# Autodesk Inventor assembly: Ensamblaje1
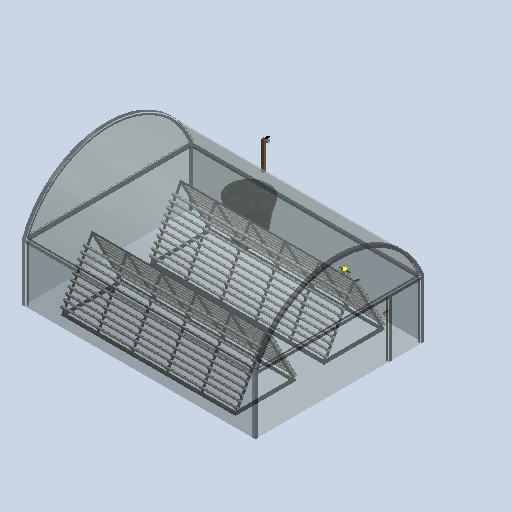
[picture p0: Inventor's stored thumbnail of the model, 512x512]
Saved by Autodesk Inventor 2026.1 (Build 301233020, 233B)
## iProperties
Created: 2025-11-02
Part Number: Ensamblaje1
Document SubType Name: Assembly
Designer: PAVILION
Author: PAVILION
## Documents named in this file (12)
- C:\Users\Alejo D\Desktop\Trabajo de Grado\Modelo de Cajas Final Inventor\Invernadero\Ensamble\Ensamblaje1.iam
- C:\Users\Alejo D\Desktop\Trabajo de Grado\Modelo de Cajas Final Inventor\Invernadero\Piezas\Invernadero.ipt
- C:\Users\Alejo D\Desktop\Trabajo de Grado\Modelo de Cajas Final Inventor\Invernadero\Piezas\Torre.ipt
- C:\Users\Alejo D\Desktop\Trabajo de Grado\Modelo de Cajas Final Inventor\Invernadero\Piezas\Tubo.ipt
- C:\Users\Alejo D\Desktop\Trabajo de Grado\Modelo de Cajas Final Inventor\Caja EC Final v13\Caja EC Final.iam
- C:\Users\Alejo D\Desktop\Trabajo de Grado\Modelo de Cajas Final Inventor\Invernadero\Piezas\Tanque.ipt
- C:\Users\Alejo D\Desktop\Trabajo de Grado\Modelo de Cajas Final Inventor\Invernadero\Piezas\TapaTanque.ipt
- C:\Users\Alejo D\Desktop\Trabajo de Grado\Modelo de Cajas Final Inventor\Invernadero\Piezas\Soporte.ipt
- C:\Users\Alejo D\Desktop\Trabajo de Grado\Modelo de Cajas Final Inventor\Caja pH Final v8\Caja pH Final.iam
- C:\Users\Alejo D\Desktop\Trabajo de Grado\Modelo de Cajas Final Inventor\Caja nivel Final v5\Caja nivel Final.iam
- C:\Users\Alejo D\Desktop\Trabajo de Grado\Modelo de Cajas Final Inventor\Caja sen altura Final v4\Caja sen altura Final.iam
- C:\Users\Alejo D\Desktop\Trabajo de Grado\Modelo de Cajas Final Inventor\Caja Princi FInal v7\Caja Princi FInal.iam
## Components (54 placed, 11 different names)
1. Torre:1 — Insertar:1, Coincidencia:1, Coincidencia:2, Insertar:2, Insertar:3, Coincidencia:3, Coincidencia:4, Coincidencia:5, Insertar:4, Insertar:5, Insertar:6, Insertar:7, Insertar:8, Insertar:9, Insertar:10, Insertar:11, Insertar:12, Insertar:13, Insertar:14, Insertar:15, Nivelación:1, Nivelación:2, Coincidencia:11, Nivelación:3, Coincidencia:12, Coincidencia:13, Coincidencia:14, Coincidencia:17, Coincidencia:18, Coincidencia:19, Coincidencia:20
2. Tubo:3 — Insertar:1
3. Tubo:4 — Coincidencia:1
4. Tubo:5 — Coincidencia:2
5. Tubo:6 — Insertar:2
6. Tubo:7 — Insertar:3
7. Tubo:8 — Coincidencia:3
8. Tubo:9 — Coincidencia:4
9. Tubo:10 — Coincidencia:5
10. Tubo:11 — Insertar:4
11. Tubo:12 — Insertar:5
12. Tubo:13 — Insertar:6
13. Tubo:14 — Insertar:7
14. Tubo:15 — Insertar:8
15. Tubo:16 — Insertar:9
16. Tubo:17 — Insertar:10
17. Tubo:18 — Insertar:11
18. Tubo:19 — Insertar:12
19. Tubo:20 — Insertar:13
20. Tubo:21 — Insertar:14
21. Tubo:22 — Insertar:15
22. Torre:2 — Nivelación:1, Nivelación:2, Coincidencia:11
23. Tubo:23
24. Tubo:24
25. Tubo:25
26. Tubo:26
27. Tubo:27
28. Tubo:28
29. Tubo:29
30. Tubo:30
31. Tubo:31
32. Tubo:32
33. Tubo:33
34. Tubo:34
35. Tubo:35
36. Tubo:36
37. Tubo:37
38. Tubo:38
39. Tubo:39
40. Tubo:40
41. Tubo:41
42. Tubo:42
43. Invernadero:1 — Nivelación:3, Coincidencia:12, Coincidencia:13, Coincidencia:24, Coincidencia:25, Coincidencia:26
44. Caja EC Final:1 [sub-assembly] — Coincidencia:14
45. Tanque:1 — Coincidencia:15
46. TapaTanque:1 — Coincidencia:15, Coincidencia:16
47. Soporte:1 — Coincidencia:16, Coincidencia:21, Coincidencia:22, Coincidencia:23
48. Caja pH Final:1 [sub-assembly] — Coincidencia:17
49. Caja nivel Final:1 [sub-assembly] — Coincidencia:18, Coincidencia:19, Coincidencia:20
50. Caja sen altura Final:1 [sub-assembly] — Coincidencia:21, Coincidencia:22, Coincidencia:23
51. Caja nivel Final:2 [sub-assembly]
52. Caja pH Final:2 [sub-assembly]
53. Caja EC Final:2 [sub-assembly]
54. Caja Princi FInal:1 [sub-assembly] — Coincidencia:24, Coincidencia:25, Coincidencia:26
## Relationships (59: Insert 30, Mate 26, Flush 3)
- Insertar:1 (-6050 mm): Torre:1 ↔ Tubo:3
- Coincidencia:1 [Mate] (-6050 mm): Torre:1 ↔ Tubo:4
- Coincidencia:2 [Mate] (6050 mm): Torre:1 ↔ Tubo:5
- Insertar:2 (-6050 mm): Torre:1 ↔ Tubo:6
- Insertar:3 (-6050 mm): Torre:1 ↔ Tubo:7
- Coincidencia:3 [Mate] (-6050 mm): Torre:1 ↔ Tubo:8
- Coincidencia:4 [Mate] (-6050 mm): Torre:1 ↔ Tubo:9
- Coincidencia:5 [Mate] (-6050 mm): Torre:1 ↔ Tubo:10
- Insertar:4 (-6050 mm): Torre:1 ↔ Tubo:11
- Insertar:5 (-6050 mm): Torre:1 ↔ Tubo:12
- Insertar:6 (-6050 mm): Torre:1 ↔ Tubo:13
- Insertar:7 (-6050 mm): Torre:1 ↔ Tubo:14
- Insertar:8 (-6050 mm): Torre:1 ↔ Tubo:15
- Insertar:9 (-6050 mm): Torre:1 ↔ Tubo:16
- Insertar:10 (-6050 mm): Torre:1 ↔ Tubo:17
- Insertar:11 (-6050 mm): Torre:1 ↔ Tubo:18
- Insertar:12 (-6050 mm): Torre:1 ↔ Tubo:19
- Insertar:13 (-6050 mm): Torre:1 ↔ Tubo:20
- Insertar:14 (-6050 mm): Torre:1 ↔ Tubo:21
- Insertar:15 (-6050 mm): Torre:1 ↔ Tubo:22
- [Insert] (-6050 mm): Torre:2 ↔ Tubo:23
- [Mate] (-6050 mm): Torre:2 ↔ Tubo:24
- [Mate] (6050 mm): Torre:2 ↔ Tubo:25
- [Insert] (-6050 mm): Torre:2 ↔ Tubo:26
- [Insert] (-6050 mm): Torre:2 ↔ Tubo:27
- [Mate] (-6050 mm): Torre:2 ↔ Tubo:28
- [Mate] (-6050 mm): Torre:2 ↔ Tubo:29
- [Mate] (-6050 mm): Torre:2 ↔ Tubo:30
- [Insert] (-6050 mm): Torre:2 ↔ Tubo:31
- [Insert] (-6050 mm): Torre:2 ↔ Tubo:32
- [Insert] (-6050 mm): Torre:2 ↔ Tubo:33
- [Insert] (-6050 mm): Torre:2 ↔ Tubo:34
- [Insert] (-6050 mm): Torre:2 ↔ Tubo:35
- [Insert] (-6050 mm): Torre:2 ↔ Tubo:36
- [Insert] (-6050 mm): Torre:2 ↔ Tubo:37
- [Insert] (-6050 mm): Torre:2 ↔ Tubo:38
- [Insert] (-6050 mm): Torre:2 ↔ Tubo:39
- [Insert] (-6050 mm): Torre:2 ↔ Tubo:40
- [Insert] (-6050 mm): Torre:2 ↔ Tubo:41
- [Insert] (-6050 mm): Torre:2 ↔ Tubo:42
- Nivelación:1 [Flush]: Torre:1 ↔ Torre:2
- Nivelación:2 [Flush]: Torre:1 ↔ Torre:2
- Coincidencia:11 [Mate] (950 mm): Torre:1 ↔ Torre:2
- Nivelación:3 [Flush]: Torre:1 ↔ Invernadero:1
- Coincidencia:12 [Mate] (1000 mm): Torre:1 ↔ Invernadero:1
- Coincidencia:13 [Mate] (270 mm): Torre:1 ↔ Invernadero:1
- Coincidencia:14 [Mate]: Torre:1 ↔ Caja EC Final:1
- Coincidencia:15 [Mate]: Tanque:1 ↔ TapaTanque:1
- Coincidencia:16 [Mate]: TapaTanque:1 ↔ Soporte:1
- Coincidencia:17 [Mate]: Torre:1 ↔ Caja pH Final:1
- Coincidencia:18 [Mate]: Torre:1 ↔ Caja nivel Final:1
- Coincidencia:19 [Mate]: Torre:1 ↔ Caja nivel Final:1
- Coincidencia:20 [Mate]: Torre:1 ↔ Caja nivel Final:1
- Coincidencia:21 [Mate]: Soporte:1 ↔ Caja sen altura Final:1
- Coincidencia:22 [Mate]: Soporte:1 ↔ Caja sen altura Final:1
- Coincidencia:23 [Mate]: Soporte:1 ↔ Caja sen altura Final:1
- Coincidencia:24 [Mate]: Invernadero:1 ↔ Caja Princi FInal:1
- Coincidencia:25 [Mate]: Invernadero:1 ↔ Caja Princi FInal:1
- Coincidencia:26 [Mate]: Invernadero:1 ↔ Caja Princi FInal:1
